# Autodesk Inventor assembly: ASY ДМФГиД 01010 крышка галка ПВГ
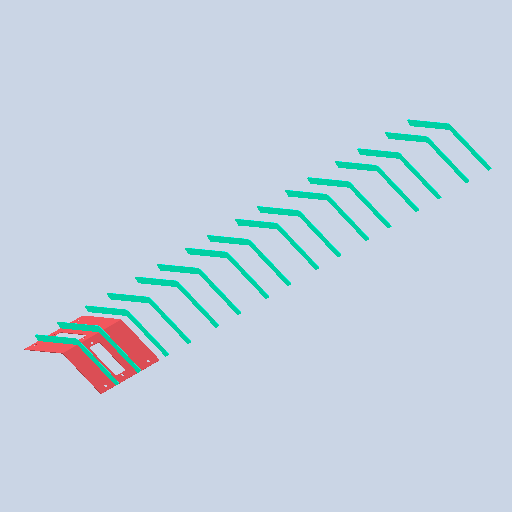
[picture p0: Inventor's stored thumbnail of the model, 512x512]
Saved by Autodesk Inventor 2024.2 (Build 282272000, 272)
## iProperties
Created: 2024-04-30
Part Number: ASY ДМФГиД 01010 крышка галка ПВГ
Document SubType Name: Assembly
Designer: admin
Author: admin
## Documents named in this file (3)
- C:\Users\pokla\Documents\Inventor\ДФО\ДМФ\DMF-Disk-Micro-Filter-main 12.05.24 12-39\Пробный вал Глеб\ASY ДМФГиД 01010 крышка галка ПВГ.iam
- C:\Users\pokla\Documents\Inventor\ДФО\ДМФ\DMF-Disk-Micro-Filter-main 12.05.24 12-39\Пробный вал Глеб\ДМС 100 Барабан Лист №1 ПВГ.ipt
- C:\Users\pokla\Documents\Inventor\ДФО\ДМФ\DMF-Disk-Micro-Filter-main 12.05.24 12-39\Пробный вал Глеб\ДМС 104 Сектор кольца усилителя барабана_CPY ПВГ.ipt
## Components (17 placed, 2 different names)
1. ДМС 100 Барабан Лист №1 ПВГ:1 — Mate:1, Mate:2, Flush:1
2. ДМС 104 Сектор кольца усилителя барабана_CPY ПВГ:2 — Rigid:1
3. ДМС 104 Сектор кольца усилителя барабана_CPY ПВГ:1 — Mate:1, Mate:2, Rigid:1
4. ДМС 104 Сектор кольца усилителя барабана_CPY ПВГ:3
5. ДМС 104 Сектор кольца усилителя барабана_CPY ПВГ:4
6. ДМС 104 Сектор кольца усилителя барабана_CPY ПВГ:5
7. ДМС 104 Сектор кольца усилителя барабана_CPY ПВГ:6
8. ДМС 104 Сектор кольца усилителя барабана_CPY ПВГ:7
9. ДМС 104 Сектор кольца усилителя барабана_CPY ПВГ:8
10. ДМС 104 Сектор кольца усилителя барабана_CPY ПВГ:9
11. ДМС 104 Сектор кольца усилителя барабана_CPY ПВГ:10
12. ДМС 104 Сектор кольца усилителя барабана_CPY ПВГ:11
13. ДМС 104 Сектор кольца усилителя барабана_CPY ПВГ:12
14. ДМС 104 Сектор кольца усилителя барабана_CPY ПВГ:13
15. ДМС 104 Сектор кольца усилителя барабана_CPY ПВГ:14
16. ДМС 104 Сектор кольца усилителя барабана_CPY ПВГ:15 — Flush:1
17. ДМС 104 Сектор кольца усилителя барабана_CPY ПВГ:16
## Component patterns: (8 elements, first: ДМС 104 Сектор кольца усилителя барабана_CPY ПВГ:2 + ДМС 104 Сектор кольца усилителя барабана_CPY ПВГ:1)
## Relationships (4: Mate 2, WeldJoint 1, Flush 1)
- Mate:1: ДМС 100 Барабан Лист №1 ПВГ:1 ↔ ДМС 104 Сектор кольца усилителя барабана_CPY ПВГ:1
- Mate:2: ДМС 100 Барабан Лист №1 ПВГ:1 ↔ ДМС 104 Сектор кольца усилителя барабана_CPY ПВГ:1
- Rigid:1 [WeldJoint] (108 mm): ДМС 104 Сектор кольца усилителя барабана_CPY ПВГ:2 ↔ ДМС 104 Сектор кольца усилителя барабана_CPY ПВГ:1
- Flush:1 (29 mm): ДМС 100 Барабан Лист №1 ПВГ:1 ↔ ДМС 104 Сектор кольца усилителя барабана_CPY ПВГ:15
